# Autodesk Inventor assembly: SIDE REDUCTION
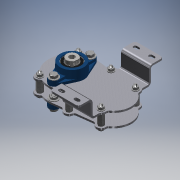
[picture p0: Inventor's stored thumbnail of the model, 180x180]
Saved by Autodesk Inventor 2017 (Build 210142000, 142)
## iProperties
Part Number: SIDE REDUCTION
Material: Genérico
Document SubType Name: Assembly
Designer: Cristian
Author: Cristian
## Documents named in this file (11)
- C:\Users\Cristian\Desktop\DISEÑO\CNCO PLASMA CAD\SIDE REDUCTION\SIDE REDUCTION.iam
- C:\Users\Cristian\Desktop\DISEÑO\CNCO PLASMA CAD\SIDE REDUCTION\STEEL SIDE REDUCTION FRONT PLATE.ipt
- C:\Users\Cristian\Desktop\DISEÑO\CNCO PLASMA CAD\SIDE REDUCTION\1-2 HEX_1 1-8 LNG _1-4 THR_STANDOFF.ipt
- C:\Users\Cristian\Desktop\DISEÑO\CNCO PLASMA CAD\SIDE REDUCTION\STEEL SIDE REDUCTION COUNTER PLATE.ipt
- C:\Users\Cristian\Desktop\DISEÑO\CNCO PLASMA CAD\SIDE REDUCTION\1-4 - 20 STEEL HEX CAP SCREW.ipt
- C:\Users\Cristian\Desktop\DISEÑO\CNCO PLASMA CAD\SIDE REDUCTION\1-4 IN SCREW STEEL FLAT WASHER.ipt
- C:\Users\Cristian\Desktop\DISEÑO\CNCO PLASMA CAD\SIDE REDUCTION\1-4 - 20 SCREW STEEL HEX NUT.ipt
- C:\Users\Cristian\Desktop\DISEÑO\CNCO PLASMA CAD\SIDE REDUCTION\UCFL201-08 TWO-BOLT FLANGE BEARING.ipt
- C:\Users\Cristian\Desktop\DISEÑO\CNCO PLASMA CAD\SIDE REDUCTION\3-8 IN SCREW STEEL FLAT WASHER.ipt
- C:\Users\Cristian\Desktop\DISEÑO\CNCO PLASMA CAD\SIDE REDUCTION\3-8 - 16 SCREW STEEL THIN HEX NUT.ipt
- C:\Users\Cristian\Desktop\DISEÑO\CNCO PLASMA CAD\SIDE REDUCTION\3-8 - 16 STEEL HEX CAP SCREW.ipt
## Components (50 placed, 10 different names)
1. STEEL SIDE REDUCTION FRONT PLATE:1 — Coincidencia:1, Coincidencia:2, Coincidencia:3, Coincidencia:4, Coincidencia:5, Coincidencia:6, Coincidencia:7, Coincidencia:8, Coincidencia:9, Coincidencia:10, Coincidencia:11, Coincidencia:12, Coincidencia:40, Coincidencia:41, Coincidencia:42, Coincidencia:43, Coincidencia:44, Coincidencia:45, Coincidencia:46, Coincidencia:47, Coincidencia:48, Coincidencia:49, Coincidencia:50, Coincidencia:51, Coincidencia:53, Coincidencia:55, Coincidencia:57, Coincidencia:59, Coincidencia:61, Coincidencia:63, Coincidencia:64, Coincidencia:65, Coincidencia:66, Coincidencia:88, Coincidencia:89, Coincidencia:90, Coincidencia:91, Coincidencia:92, Coincidencia:93, Coincidencia:95, Coincidencia:97, Coincidencia:98, Coincidencia:100
2. STEEL SIDE REDUCTION COUNTER PLATE:1 — Coincidencia:13, Coincidencia:14, Coincidencia:15, Coincidencia:16, Coincidencia:17, Coincidencia:18, Coincidencia:20, Coincidencia:21, Coincidencia:22, Coincidencia:24, Coincidencia:25, Coincidencia:26, Coincidencia:27, Coincidencia:28, Coincidencia:29, Coincidencia:30, Coincidencia:31, Coincidencia:32, Coincidencia:34, Coincidencia:35, Coincidencia:36, Coincidencia:38, Coincidencia:67, Coincidencia:68, Coincidencia:69, Coincidencia:71, Coincidencia:74, Coincidencia:75, Coincidencia:76, Coincidencia:77, Coincidencia:79, Coincidencia:81, Coincidencia:83
3. UCFL201-08 TWO-BOLT FLANGE BEARING:1 — Coincidencia:64, Coincidencia:65, Coincidencia:66, Coincidencia:86, Coincidencia:87
4. UCFL201-08 TWO-BOLT FLANGE BEARING:2 — Coincidencia:67, Coincidencia:68, Coincidencia:69, Coincidencia:70, Coincidencia:72, Coincidencia:73, Coincidencia:85
5. 1-2 HEX_1 1-8 LNG _1-4 THR_STANDOFF:1 — Coincidencia:3, Coincidencia:4
6. 1-2 HEX_1 1-8 LNG _1-4 THR_STANDOFF:2 — Coincidencia:7, Coincidencia:8, Coincidencia:14
7. 1-2 HEX_1 1-8 LNG _1-4 THR_STANDOFF:3 — Coincidencia:11, Coincidencia:12
8. 1-2 HEX_1 1-8 LNG _1-4 THR_STANDOFF:4 — Coincidencia:9, Coincidencia:10
9. 1-2 HEX_1 1-8 LNG _1-4 THR_STANDOFF:5 — Coincidencia:5, Coincidencia:6, Coincidencia:15
10. 1-2 HEX_1 1-8 LNG _1-4 THR_STANDOFF:6 — Coincidencia:1, Coincidencia:2, Coincidencia:13
11. 1-4 - 20 STEEL HEX CAP SCREW:1 — Coincidencia:22, Coincidencia:23
12. 1-4 - 20 STEEL HEX CAP SCREW:2 — Coincidencia:32, Coincidencia:33
13. 1-4 - 20 STEEL HEX CAP SCREW:3 — Coincidencia:16, Coincidencia:19
14. 1-4 - 20 STEEL HEX CAP SCREW:4 — Coincidencia:36, Coincidencia:37
15. 1-4 - 20 STEEL HEX CAP SCREW:5 — Coincidencia:38, Coincidencia:39
16. 1-4 - 20 STEEL HEX CAP SCREW:6 — Coincidencia:34, Coincidencia:35
17. 1-4 IN SCREW STEEL FLAT WASHER:7 — Coincidencia:42, Coincidencia:43, Coincidencia:52
18. 1-4 IN SCREW STEEL FLAT WASHER:8 — Coincidencia:48, Coincidencia:49, Coincidencia:58
19. 1-4 IN SCREW STEEL FLAT WASHER:9 — Coincidencia:50, Coincidencia:51, Coincidencia:60
20. 1-4 IN SCREW STEEL FLAT WASHER:10 — Coincidencia:44, Coincidencia:45, Coincidencia:62
21. 1-4 IN SCREW STEEL FLAT WASHER:11 — Coincidencia:40, Coincidencia:41, Coincidencia:54
22. 1-4 IN SCREW STEEL FLAT WASHER:12 — Coincidencia:46, Coincidencia:47, Coincidencia:56
23. 1-4 IN SCREW STEEL FLAT WASHER:1 — Coincidencia:20, Coincidencia:21, Coincidencia:23
24. 1-4 IN SCREW STEEL FLAT WASHER:2 — Coincidencia:24, Coincidencia:25, Coincidencia:33
25. 1-4 IN SCREW STEEL FLAT WASHER:3 — Coincidencia:30, Coincidencia:31, Coincidencia:39
26. 1-4 IN SCREW STEEL FLAT WASHER:4 — Coincidencia:28, Coincidencia:29, Coincidencia:37
27. 1-4 IN SCREW STEEL FLAT WASHER:5 — Coincidencia:26, Coincidencia:27
28. 1-4 IN SCREW STEEL FLAT WASHER:6 — Coincidencia:17, Coincidencia:18, Coincidencia:19
29. 1-4 - 20 SCREW STEEL HEX NUT:1 — Coincidencia:58, Coincidencia:59
30. 1-4 - 20 SCREW STEEL HEX NUT:2 — Coincidencia:60, Coincidencia:61
31. 1-4 - 20 SCREW STEEL HEX NUT:3 — Coincidencia:56, Coincidencia:57
32. 1-4 - 20 SCREW STEEL HEX NUT:4 — Coincidencia:62, Coincidencia:63
33. 1-4 - 20 SCREW STEEL HEX NUT:5 — Coincidencia:52, Coincidencia:53
34. 1-4 - 20 SCREW STEEL HEX NUT:6 — Coincidencia:54, Coincidencia:55
35. 3-8 IN SCREW STEEL FLAT WASHER:5 — Coincidencia:86, Coincidencia:92, Coincidencia:94
36. 3-8 IN SCREW STEEL FLAT WASHER:6 — Coincidencia:88, Coincidencia:91, Coincidencia:101
37. 3-8 IN SCREW STEEL FLAT WASHER:7 — Coincidencia:87, Coincidencia:93, Coincidencia:96
38. 3-8 IN SCREW STEEL FLAT WASHER:8 — Coincidencia:89, Coincidencia:90, Coincidencia:99
39. 3-8 IN SCREW STEEL FLAT WASHER:1 — Coincidencia:72, Coincidencia:73, Coincidencia:84
40. 3-8 IN SCREW STEEL FLAT WASHER:2 — Coincidencia:70, Coincidencia:71, Coincidencia:82
41. 3-8 IN SCREW STEEL FLAT WASHER:3 — Coincidencia:76, Coincidencia:77, Coincidencia:80
42. 3-8 IN SCREW STEEL FLAT WASHER:4 — Coincidencia:74, Coincidencia:75, Coincidencia:78
43. 3-8 - 16 STEEL HEX CAP SCREW:1 — Coincidencia:84, Coincidencia:85
44. 3-8 - 16 STEEL HEX CAP SCREW:2 — Coincidencia:82, Coincidencia:83
45. 3-8 - 16 STEEL HEX CAP SCREW:3 — Coincidencia:96, Coincidencia:97
46. 3-8 - 16 STEEL HEX CAP SCREW:4 — Coincidencia:94, Coincidencia:95
47. 3-8 - 16 SCREW STEEL THIN HEX NUT:3 — Coincidencia:100, Coincidencia:101
48. 3-8 - 16 SCREW STEEL THIN HEX NUT:1 — Coincidencia:78, Coincidencia:79
49. 3-8 - 16 SCREW STEEL THIN HEX NUT:2 — Coincidencia:80, Coincidencia:81
50. 3-8 - 16 SCREW STEEL THIN HEX NUT:4 — Coincidencia:98, Coincidencia:99
## Relationships (101: Mate 101)
- Coincidencia:1 [Mate]: STEEL SIDE REDUCTION FRONT PLATE:1 ↔ 1-2 HEX_1 1-8 LNG _1-4 THR_STANDOFF:6
- Coincidencia:2 [Mate]: STEEL SIDE REDUCTION FRONT PLATE:1 ↔ 1-2 HEX_1 1-8 LNG _1-4 THR_STANDOFF:6
- Coincidencia:3 [Mate]: STEEL SIDE REDUCTION FRONT PLATE:1 ↔ 1-2 HEX_1 1-8 LNG _1-4 THR_STANDOFF:1
- Coincidencia:4 [Mate]: STEEL SIDE REDUCTION FRONT PLATE:1 ↔ 1-2 HEX_1 1-8 LNG _1-4 THR_STANDOFF:1
- Coincidencia:5 [Mate]: STEEL SIDE REDUCTION FRONT PLATE:1 ↔ 1-2 HEX_1 1-8 LNG _1-4 THR_STANDOFF:5
- Coincidencia:6 [Mate]: STEEL SIDE REDUCTION FRONT PLATE:1 ↔ 1-2 HEX_1 1-8 LNG _1-4 THR_STANDOFF:5
- Coincidencia:7 [Mate]: STEEL SIDE REDUCTION FRONT PLATE:1 ↔ 1-2 HEX_1 1-8 LNG _1-4 THR_STANDOFF:2
- Coincidencia:8 [Mate]: STEEL SIDE REDUCTION FRONT PLATE:1 ↔ 1-2 HEX_1 1-8 LNG _1-4 THR_STANDOFF:2
- Coincidencia:9 [Mate]: STEEL SIDE REDUCTION FRONT PLATE:1 ↔ 1-2 HEX_1 1-8 LNG _1-4 THR_STANDOFF:4
- Coincidencia:10 [Mate]: STEEL SIDE REDUCTION FRONT PLATE:1 ↔ 1-2 HEX_1 1-8 LNG _1-4 THR_STANDOFF:4
- Coincidencia:11 [Mate]: STEEL SIDE REDUCTION FRONT PLATE:1 ↔ 1-2 HEX_1 1-8 LNG _1-4 THR_STANDOFF:3
- Coincidencia:12 [Mate]: STEEL SIDE REDUCTION FRONT PLATE:1 ↔ 1-2 HEX_1 1-8 LNG _1-4 THR_STANDOFF:3
- Coincidencia:13 [Mate]: STEEL SIDE REDUCTION COUNTER PLATE:1 ↔ 1-2 HEX_1 1-8 LNG _1-4 THR_STANDOFF:6
- Coincidencia:14 [Mate]: STEEL SIDE REDUCTION COUNTER PLATE:1 ↔ 1-2 HEX_1 1-8 LNG _1-4 THR_STANDOFF:2
- Coincidencia:15 [Mate]: STEEL SIDE REDUCTION COUNTER PLATE:1 ↔ 1-2 HEX_1 1-8 LNG _1-4 THR_STANDOFF:5
- Coincidencia:16 [Mate]: STEEL SIDE REDUCTION COUNTER PLATE:1 ↔ 1-4 - 20 STEEL HEX CAP SCREW:3
- Coincidencia:17 [Mate]: STEEL SIDE REDUCTION COUNTER PLATE:1 ↔ 1-4 IN SCREW STEEL FLAT WASHER:6
- Coincidencia:18 [Mate]: STEEL SIDE REDUCTION COUNTER PLATE:1 ↔ 1-4 IN SCREW STEEL FLAT WASHER:6
- Coincidencia:19 [Mate]: 1-4 - 20 STEEL HEX CAP SCREW:3 ↔ 1-4 IN SCREW STEEL FLAT WASHER:6
- Coincidencia:20 [Mate]: STEEL SIDE REDUCTION COUNTER PLATE:1 ↔ 1-4 IN SCREW STEEL FLAT WASHER:1
- Coincidencia:21 [Mate]: STEEL SIDE REDUCTION COUNTER PLATE:1 ↔ 1-4 IN SCREW STEEL FLAT WASHER:1
- Coincidencia:22 [Mate]: STEEL SIDE REDUCTION COUNTER PLATE:1 ↔ 1-4 - 20 STEEL HEX CAP SCREW:1
- Coincidencia:23 [Mate]: 1-4 - 20 STEEL HEX CAP SCREW:1 ↔ 1-4 IN SCREW STEEL FLAT WASHER:1
- Coincidencia:24 [Mate]: STEEL SIDE REDUCTION COUNTER PLATE:1 ↔ 1-4 IN SCREW STEEL FLAT WASHER:2
- Coincidencia:25 [Mate]: STEEL SIDE REDUCTION COUNTER PLATE:1 ↔ 1-4 IN SCREW STEEL FLAT WASHER:2
- Coincidencia:26 [Mate]: STEEL SIDE REDUCTION COUNTER PLATE:1 ↔ 1-4 IN SCREW STEEL FLAT WASHER:5
- Coincidencia:27 [Mate]: STEEL SIDE REDUCTION COUNTER PLATE:1 ↔ 1-4 IN SCREW STEEL FLAT WASHER:5
- Coincidencia:28 [Mate]: STEEL SIDE REDUCTION COUNTER PLATE:1 ↔ 1-4 IN SCREW STEEL FLAT WASHER:4
- Coincidencia:29 [Mate]: STEEL SIDE REDUCTION COUNTER PLATE:1 ↔ 1-4 IN SCREW STEEL FLAT WASHER:4
- Coincidencia:30 [Mate]: STEEL SIDE REDUCTION COUNTER PLATE:1 ↔ 1-4 IN SCREW STEEL FLAT WASHER:3
- Coincidencia:31 [Mate]: STEEL SIDE REDUCTION COUNTER PLATE:1 ↔ 1-4 IN SCREW STEEL FLAT WASHER:3
- Coincidencia:32 [Mate]: STEEL SIDE REDUCTION COUNTER PLATE:1 ↔ 1-4 - 20 STEEL HEX CAP SCREW:2
- Coincidencia:33 [Mate]: 1-4 - 20 STEEL HEX CAP SCREW:2 ↔ 1-4 IN SCREW STEEL FLAT WASHER:2
- Coincidencia:34 [Mate]: STEEL SIDE REDUCTION COUNTER PLATE:1 ↔ 1-4 - 20 STEEL HEX CAP SCREW:6
- Coincidencia:35 [Mate]: STEEL SIDE REDUCTION COUNTER PLATE:1 ↔ 1-4 - 20 STEEL HEX CAP SCREW:6
- Coincidencia:36 [Mate]: STEEL SIDE REDUCTION COUNTER PLATE:1 ↔ 1-4 - 20 STEEL HEX CAP SCREW:4
- Coincidencia:37 [Mate]: 1-4 - 20 STEEL HEX CAP SCREW:4 ↔ 1-4 IN SCREW STEEL FLAT WASHER:4
- Coincidencia:38 [Mate]: STEEL SIDE REDUCTION COUNTER PLATE:1 ↔ 1-4 - 20 STEEL HEX CAP SCREW:5
- Coincidencia:39 [Mate]: 1-4 - 20 STEEL HEX CAP SCREW:5 ↔ 1-4 IN SCREW STEEL FLAT WASHER:3
- Coincidencia:40 [Mate]: STEEL SIDE REDUCTION FRONT PLATE:1 ↔ 1-4 IN SCREW STEEL FLAT WASHER:11
- Coincidencia:41 [Mate]: STEEL SIDE REDUCTION FRONT PLATE:1 ↔ 1-4 IN SCREW STEEL FLAT WASHER:11
- Coincidencia:42 [Mate]: STEEL SIDE REDUCTION FRONT PLATE:1 ↔ 1-4 IN SCREW STEEL FLAT WASHER:7
- Coincidencia:43 [Mate]: STEEL SIDE REDUCTION FRONT PLATE:1 ↔ 1-4 IN SCREW STEEL FLAT WASHER:7
- Coincidencia:44 [Mate]: STEEL SIDE REDUCTION FRONT PLATE:1 ↔ 1-4 IN SCREW STEEL FLAT WASHER:10
- Coincidencia:45 [Mate]: STEEL SIDE REDUCTION FRONT PLATE:1 ↔ 1-4 IN SCREW STEEL FLAT WASHER:10
- Coincidencia:46 [Mate]: STEEL SIDE REDUCTION FRONT PLATE:1 ↔ 1-4 IN SCREW STEEL FLAT WASHER:12
- Coincidencia:47 [Mate]: STEEL SIDE REDUCTION FRONT PLATE:1 ↔ 1-4 IN SCREW STEEL FLAT WASHER:12
- Coincidencia:48 [Mate]: STEEL SIDE REDUCTION FRONT PLATE:1 ↔ 1-4 IN SCREW STEEL FLAT WASHER:8
- Coincidencia:49 [Mate]: STEEL SIDE REDUCTION FRONT PLATE:1 ↔ 1-4 IN SCREW STEEL FLAT WASHER:8
- Coincidencia:50 [Mate]: STEEL SIDE REDUCTION FRONT PLATE:1 ↔ 1-4 IN SCREW STEEL FLAT WASHER:9
- Coincidencia:51 [Mate]: STEEL SIDE REDUCTION FRONT PLATE:1 ↔ 1-4 IN SCREW STEEL FLAT WASHER:9
- Coincidencia:52 [Mate]: 1-4 IN SCREW STEEL FLAT WASHER:7 ↔ 1-4 - 20 SCREW STEEL HEX NUT:5
- Coincidencia:53 [Mate]: STEEL SIDE REDUCTION FRONT PLATE:1 ↔ 1-4 - 20 SCREW STEEL HEX NUT:5
- Coincidencia:54 [Mate]: 1-4 IN SCREW STEEL FLAT WASHER:11 ↔ 1-4 - 20 SCREW STEEL HEX NUT:6
- Coincidencia:55 [Mate]: STEEL SIDE REDUCTION FRONT PLATE:1 ↔ 1-4 - 20 SCREW STEEL HEX NUT:6
- Coincidencia:56 [Mate]: 1-4 IN SCREW STEEL FLAT WASHER:12 ↔ 1-4 - 20 SCREW STEEL HEX NUT:3
- Coincidencia:57 [Mate]: STEEL SIDE REDUCTION FRONT PLATE:1 ↔ 1-4 - 20 SCREW STEEL HEX NUT:3
- Coincidencia:58 [Mate]: 1-4 IN SCREW STEEL FLAT WASHER:8 ↔ 1-4 - 20 SCREW STEEL HEX NUT:1
- Coincidencia:59 [Mate]: STEEL SIDE REDUCTION FRONT PLATE:1 ↔ 1-4 - 20 SCREW STEEL HEX NUT:1
- Coincidencia:60 [Mate]: 1-4 IN SCREW STEEL FLAT WASHER:9 ↔ 1-4 - 20 SCREW STEEL HEX NUT:2
- Coincidencia:61 [Mate]: STEEL SIDE REDUCTION FRONT PLATE:1 ↔ 1-4 - 20 SCREW STEEL HEX NUT:2
- Coincidencia:62 [Mate]: 1-4 IN SCREW STEEL FLAT WASHER:10 ↔ 1-4 - 20 SCREW STEEL HEX NUT:4
- Coincidencia:63 [Mate]: STEEL SIDE REDUCTION FRONT PLATE:1 ↔ 1-4 - 20 SCREW STEEL HEX NUT:4
- Coincidencia:64 [Mate]: STEEL SIDE REDUCTION FRONT PLATE:1 ↔ UCFL201-08 TWO-BOLT FLANGE BEARING:1
- Coincidencia:65 [Mate]: STEEL SIDE REDUCTION FRONT PLATE:1 ↔ UCFL201-08 TWO-BOLT FLANGE BEARING:1
- Coincidencia:66 [Mate]: STEEL SIDE REDUCTION FRONT PLATE:1 ↔ UCFL201-08 TWO-BOLT FLANGE BEARING:1
- Coincidencia:67 [Mate]: STEEL SIDE REDUCTION COUNTER PLATE:1 ↔ UCFL201-08 TWO-BOLT FLANGE BEARING:2
- Coincidencia:68 [Mate]: STEEL SIDE REDUCTION COUNTER PLATE:1 ↔ UCFL201-08 TWO-BOLT FLANGE BEARING:2
- Coincidencia:69 [Mate]: STEEL SIDE REDUCTION COUNTER PLATE:1 ↔ UCFL201-08 TWO-BOLT FLANGE BEARING:2
- Coincidencia:70 [Mate]: UCFL201-08 TWO-BOLT FLANGE BEARING:2 ↔ 3-8 IN SCREW STEEL FLAT WASHER:2
- Coincidencia:71 [Mate]: STEEL SIDE REDUCTION COUNTER PLATE:1 ↔ 3-8 IN SCREW STEEL FLAT WASHER:2
- Coincidencia:72 [Mate]: UCFL201-08 TWO-BOLT FLANGE BEARING:2 ↔ 3-8 IN SCREW STEEL FLAT WASHER:1
- Coincidencia:73 [Mate]: UCFL201-08 TWO-BOLT FLANGE BEARING:2 ↔ 3-8 IN SCREW STEEL FLAT WASHER:1
- Coincidencia:74 [Mate]: STEEL SIDE REDUCTION COUNTER PLATE:1 ↔ 3-8 IN SCREW STEEL FLAT WASHER:4
- Coincidencia:75 [Mate]: STEEL SIDE REDUCTION COUNTER PLATE:1 ↔ 3-8 IN SCREW STEEL FLAT WASHER:4
- Coincidencia:76 [Mate]: STEEL SIDE REDUCTION COUNTER PLATE:1 ↔ 3-8 IN SCREW STEEL FLAT WASHER:3
- Coincidencia:77 [Mate]: STEEL SIDE REDUCTION COUNTER PLATE:1 ↔ 3-8 IN SCREW STEEL FLAT WASHER:3
- Coincidencia:78 [Mate]: 3-8 IN SCREW STEEL FLAT WASHER:4 ↔ 3-8 - 16 SCREW STEEL THIN HEX NUT:1
- Coincidencia:79 [Mate]: STEEL SIDE REDUCTION COUNTER PLATE:1 ↔ 3-8 - 16 SCREW STEEL THIN HEX NUT:1
- Coincidencia:80 [Mate]: 3-8 IN SCREW STEEL FLAT WASHER:3 ↔ 3-8 - 16 SCREW STEEL THIN HEX NUT:2
- Coincidencia:81 [Mate]: STEEL SIDE REDUCTION COUNTER PLATE:1 ↔ 3-8 - 16 SCREW STEEL THIN HEX NUT:2
- Coincidencia:82 [Mate]: 3-8 IN SCREW STEEL FLAT WASHER:2 ↔ 3-8 - 16 STEEL HEX CAP SCREW:2
- Coincidencia:83 [Mate]: STEEL SIDE REDUCTION COUNTER PLATE:1 ↔ 3-8 - 16 STEEL HEX CAP SCREW:2
- Coincidencia:84 [Mate]: 3-8 IN SCREW STEEL FLAT WASHER:1 ↔ 3-8 - 16 STEEL HEX CAP SCREW:1
- Coincidencia:85 [Mate]: UCFL201-08 TWO-BOLT FLANGE BEARING:2 ↔ 3-8 - 16 STEEL HEX CAP SCREW:1
- Coincidencia:86 [Mate]: UCFL201-08 TWO-BOLT FLANGE BEARING:1 ↔ 3-8 IN SCREW STEEL FLAT WASHER:5
- Coincidencia:87 [Mate]: UCFL201-08 TWO-BOLT FLANGE BEARING:1 ↔ 3-8 IN SCREW STEEL FLAT WASHER:7
- Coincidencia:88 [Mate]: STEEL SIDE REDUCTION FRONT PLATE:1 ↔ 3-8 IN SCREW STEEL FLAT WASHER:6
- Coincidencia:89 [Mate]: STEEL SIDE REDUCTION FRONT PLATE:1 ↔ 3-8 IN SCREW STEEL FLAT WASHER:8
- Coincidencia:90 [Mate]: STEEL SIDE REDUCTION FRONT PLATE:1 ↔ 3-8 IN SCREW STEEL FLAT WASHER:8
- Coincidencia:91 [Mate]: STEEL SIDE REDUCTION FRONT PLATE:1 ↔ 3-8 IN SCREW STEEL FLAT WASHER:6
- Coincidencia:92 [Mate]: STEEL SIDE REDUCTION FRONT PLATE:1 ↔ 3-8 IN SCREW STEEL FLAT WASHER:5
- Coincidencia:93 [Mate]: STEEL SIDE REDUCTION FRONT PLATE:1 ↔ 3-8 IN SCREW STEEL FLAT WASHER:7
- Coincidencia:94 [Mate]: 3-8 IN SCREW STEEL FLAT WASHER:5 ↔ 3-8 - 16 STEEL HEX CAP SCREW:4
- Coincidencia:95 [Mate]: STEEL SIDE REDUCTION FRONT PLATE:1 ↔ 3-8 - 16 STEEL HEX CAP SCREW:4
- Coincidencia:96 [Mate]: 3-8 IN SCREW STEEL FLAT WASHER:7 ↔ 3-8 - 16 STEEL HEX CAP SCREW:3
- Coincidencia:97 [Mate]: STEEL SIDE REDUCTION FRONT PLATE:1 ↔ 3-8 - 16 STEEL HEX CAP SCREW:3
- Coincidencia:98 [Mate]: STEEL SIDE REDUCTION FRONT PLATE:1 ↔ 3-8 - 16 SCREW STEEL THIN HEX NUT:4
- Coincidencia:99 [Mate]: 3-8 IN SCREW STEEL FLAT WASHER:8 ↔ 3-8 - 16 SCREW STEEL THIN HEX NUT:4
- Coincidencia:100 [Mate]: STEEL SIDE REDUCTION FRONT PLATE:1 ↔ 3-8 - 16 SCREW STEEL THIN HEX NUT:3
- Coincidencia:101 [Mate]: 3-8 IN SCREW STEEL FLAT WASHER:6 ↔ 3-8 - 16 SCREW STEEL THIN HEX NUT:3
